# Autodesk Inventor assembly: ZA_VK_010
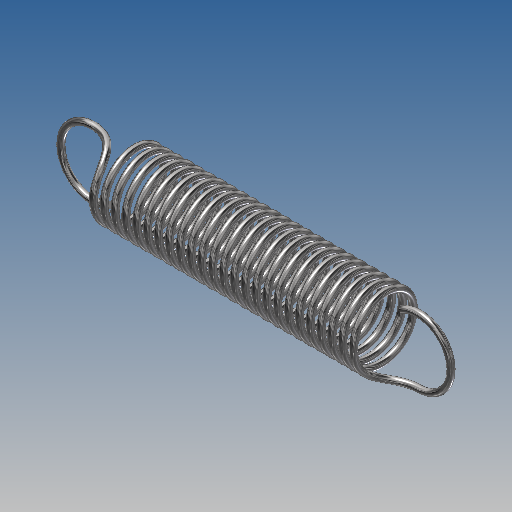
[picture p0: Inventor's stored thumbnail of the model, 512x512]
Saved by Autodesk Inventor 2017.3 (Build 213256000, 256)
## iProperties
Created: 2023-11-06
Part Number: ZA_VK_010
Document SubType Name: Assembly
Designer: Darena
Author: Darena
## Documents named in this file (3)
- D:\2_Darena\1_Soukrome\02_Inventor soukromé\Dílna RAKO3\Záhora\Pivovar KONTEJNER\S výklopným dnem\DD_KVD_001\ZA_VK_010.iam
- D:\2_Darena\1_Soukrome\02_Inventor soukromé\Dílna RAKO3\Záhora\Pivovar KONTEJNER\ZA_VK_001\ZA_VK_010_A.ipt
- D:\2_Darena\1_Soukrome\02_Inventor soukromé\Dílna RAKO3\Záhora\Pivovar KONTEJNER\ZA_VK_001\ZA_VK_010_B.ipt
## Components (2 placed, 2 different names)
1. ZA_VK_010_A:1 — Proti sobě:1, Proti sobě:2, Proti sobě:3, Proti sobě:4, Proti sobě:5, Proti sobě:6
2. ZA_VK_010_B:1 — Proti sobě:1, Proti sobě:2, Proti sobě:3
## Relationships (6: Mate 6)
- Proti sobě:1 [Mate]: ZA_VK_010_A:1 ↔ ZA_VK_010_B:1
- Proti sobě:2 [Mate]: ZA_VK_010_A:1 ↔ ZA_VK_010_B:1
- Proti sobě:3 [Mate]: ZA_VK_010_A:1 ↔ ZA_VK_010_B:1
- Proti sobě:4 [Mate]: ZA_VK_010_A:1
- Proti sobě:5 [Mate]: ZA_VK_010_A:1
- Proti sobě:6 [Mate]: ZA_VK_010_A:1
